# Autodesk Inventor assembly: Assembly10
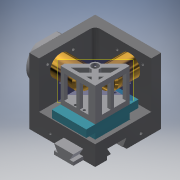
[picture p0: Inventor's stored thumbnail of the model, 180x180]
Saved by Autodesk Inventor 2018 (Build 220112000, 112)
## iProperties
Created: 2018-08-29
Part Number: Assembly10
Document SubType Name: Assembly
Designer: David
Author: David
## Documents named in this file (8)
- C:\Users\David\Documents\optoelectronics\LightSheetMicroscope\Printing\Assembly10.iam
- C:\Users\David\Documents\optoelectronics\LightSheetMicroscope\Printing\sample_holder.ipt
- C:\Users\David\Documents\optoelectronics\LightSheetMicroscope\Printing\actuator.ipt
- C:\Users\David\Documents\optoelectronics\LightSheetMicroscope\Printing\objective.ipt
- C:\Users\David\Documents\optoelectronics\LightSheetMicroscope\Printing\brain_holder.ipt
- C:\Users\David\Documents\optoelectronics\LightSheetMicroscope\Printing\modified_o_ring.ipt
- C:\Users\David\Documents\optoelectronics\LightSheetMicroscope\Printing\tester.ipt
- C:\Users\David\Documents\optoelectronics\LightSheetMicroscope\Printing\Sy_holder.ipt
## Components (8 placed, 7 different names)
1. sample_holder:1 — Mate:2, Flush:1, Mate:4, Mate:5, Flush:2, Flush:3, Mate:11, Mate:15, Mate:16, Mate:17, Mate:18, Flush:4, Flush:5
2. actuator:1 — Mate:2, Flush:1, Mate:11, Mate:12, Mate:19, Flush:6, Flush:7
3. objective:1 — Mate:4, Flush:3, Mate:13
4. objective:2 — Mate:5, Flush:2, Mate:14
5. brain_holder:1 — Mate:12, Mate:13, Mate:14
6. modified_o_ring:1 — Mate:15, Mate:16, Mate:17
7. tester:1 — Mate:18, Flush:4, Flush:5
8. Sy_holder:1 — Mate:19, Flush:6, Flush:7
## Relationships (19: Mate 12, Flush 7)
- Mate:2 (17.5 mm): sample_holder:1 ↔ actuator:1
- Flush:1 (4.5 mm): sample_holder:1 ↔ actuator:1
- Mate:4: sample_holder:1 ↔ objective:1
- Mate:5: sample_holder:1 ↔ objective:2
- Flush:2: sample_holder:1 ↔ objective:2
- Flush:3: sample_holder:1 ↔ objective:1
- Mate:11: sample_holder:1 ↔ actuator:1
- Mate:12: actuator:1 ↔ brain_holder:1
- Mate:13 (5 mm): objective:1 ↔ brain_holder:1
- Mate:14 (5 mm): objective:2 ↔ brain_holder:1
- Mate:15: sample_holder:1 ↔ modified_o_ring:1
- Mate:16: sample_holder:1 ↔ modified_o_ring:1
- Mate:17: sample_holder:1 ↔ modified_o_ring:1
- Mate:18: sample_holder:1 ↔ tester:1
- Flush:4: sample_holder:1 ↔ tester:1
- Flush:5 (9.5 mm): sample_holder:1 ↔ tester:1
- Mate:19: actuator:1 ↔ Sy_holder:1
- Flush:6: actuator:1 ↔ Sy_holder:1
- Flush:7 (9 mm): actuator:1 ↔ Sy_holder:1
